# Autodesk Inventor assembly: Latch
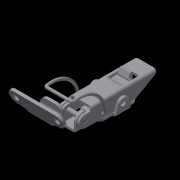
[picture p0: Inventor's stored thumbnail of the model, 180x180]
Saved by Autodesk Inventor 2014 SP1 (Build 180222100, 222)
## iProperties
Created: 2013-11-29
Part Number: Latch
Document SubType Name: Assembly
Designer: Rauhul Varma
Author: jim
Title: 6139A28.step
Description: STEP AP203
Creation Date: 2012-06-11
Sending System: SolidWorks 2009
Preprocessor: SwSTEP 2.0
Author: Rauhul Varma
## Documents named in this file (8)
- C:\Users\Rauhul Varma\Desktop\2014 Base\Latch.iam
- C:\Users\Rauhul Varma\Desktop\2014 Base\Imported Components\6139A280\1256A.ipt
- C:\Users\Rauhul Varma\Desktop\2014 Base\Imported Components\6139A280\01-600CLR.ipt
- C:\Users\Rauhul Varma\Desktop\2014 Base\Imported Components\6139A280\1256E.ipt
- C:\Users\Rauhul Varma\Desktop\2014 Base\Imported Components\6139A280\623C.ipt
- C:\Users\Rauhul Varma\Desktop\2014 Base\Imported Components\6139A280\569-2.ipt
- C:\Users\Rauhul Varma\Desktop\2014 Base\Imported Components\6139A280\RIVET.ipt
- C:\Users\Rauhul Varma\Desktop\2014 Base\Imported Components\6139A280\1256B.ipt
## Components (7 placed, 7 different names)
1. 1256A_1 — Mate:1, Mate:2, Mate:3, Mate:4, Mate:5, Mate:6, Flush:8, Angle:1
2. 01-600CLR_2 — Tangent:1, Flush:8
3. 1256E_3 — Mate:7, Mate:8, Mate:10, Mate:11, Angle:1
4. 623C_4 — Tangent:1, Mate:5, Mate:6
5. 569-2_5 — Mate:2, Mate:3
6. RIVET_6 — Mate:7, Mate:8, Mate:9
7. 1256B_7 — Mate:1, Mate:4, Mate:9, Mate:10, Mate:11
## Relationships (14: Mate 11, Tangent 1, Flush 1, Angle 1)
- Tangent:1: 01-600CLR_2 ↔ 623C_4
- Mate:1: 1256A_1 ↔ 1256B_7
- Mate:2: 1256A_1 ↔ 569-2_5
- Mate:3: 1256A_1 ↔ 569-2_5
- Mate:4 (0.6 mm): 1256A_1 ↔ 1256B_7
- Mate:5: 1256A_1 ↔ 623C_4
- Mate:6: 1256A_1 ↔ 623C_4
- Flush:8: 1256A_1 ↔ 01-600CLR_2
- Mate:7: 1256E_3 ↔ RIVET_6
- Mate:8: 1256E_3 ↔ RIVET_6
- Mate:9: RIVET_6 ↔ 1256B_7
- Mate:10: 1256E_3 ↔ 1256B_7
- Mate:11: 1256E_3 ↔ 1256B_7
- Angle:1 (180 deg): 1256A_1 ↔ 1256E_3
